# Autodesk Inventor assembly: Assembly v2
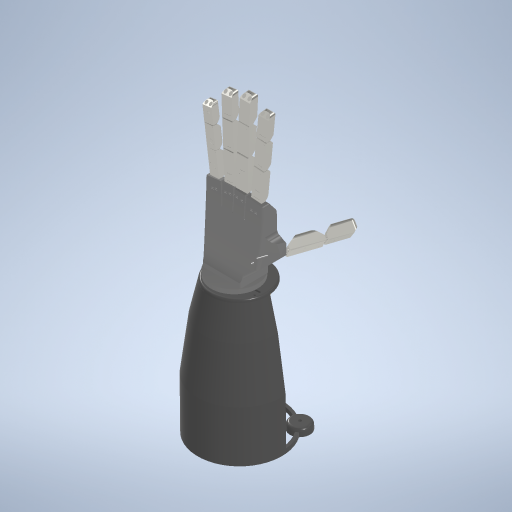
[picture p0: Inventor's stored thumbnail of the model, 512x512]
Saved by Autodesk Inventor 2024 (Build 280153000, 153)
## iProperties
Created: 2025-07-03
Part Number: Assembly v2
Document SubType Name: Assembly
Designer: Mehdi Charfeddine
Author: Mehdi Charfeddine
## Documents named in this file (15)
- C:\Users\Mehdi Charfeddine\OneDrive\Bureau\original 3d\Assembly v2.iam
- C:\Users\Mehdi Charfeddine\OneDrive\Bureau\original 3d\hand update v2.ipt
- C:\Users\Mehdi Charfeddine\OneDrive\Bureau\original 3d\update arm.ipt
- C:\Users\Mehdi Charfeddine\OneDrive\Bureau\original 3d\plaque motor.ipt
- C:\Users\Mehdi Charfeddine\OneDrive\Bureau\original 3d\finger\Daumen lower.ipt
- C:\Users\Mehdi Charfeddine\OneDrive\Bureau\original 3d\finger\Mittelfinger lower.ipt
- C:\Users\Mehdi Charfeddine\OneDrive\Bureau\original 3d\finger\Mittelfinger middle.ipt
- C:\Users\Mehdi Charfeddine\OneDrive\Bureau\original 3d\finger\Daumen upper.ipt
- C:\Users\Mehdi Charfeddine\OneDrive\Bureau\original 3d\finger\Mittelfinger upper.ipt
- C:\Users\Mehdi Charfeddine\OneDrive\Bureau\original 3d\finger\Ringfinger lower.ipt
- C:\Users\Mehdi Charfeddine\OneDrive\Bureau\original 3d\finger\Ringfinger middle.ipt
- C:\Users\Mehdi Charfeddine\OneDrive\Bureau\original 3d\finger\Ringfinger upper.ipt
- C:\Users\Mehdi Charfeddine\OneDrive\Bureau\original 3d\finger\Kleiner Finger lower.ipt
- C:\Users\Mehdi Charfeddine\OneDrive\Bureau\original 3d\finger\Kleiner Finger middle.ipt
- C:\Users\Mehdi Charfeddine\OneDrive\Bureau\original 3d\finger\Kleiner Finger upper.ipt
## Components (17 placed, 14 different names)
1. hand update v2:1 — Mate:1, Mate:3, Mate:4, Mate:8, Mate:10, Mate:14
2. update arm:1 — Mate:1, Mate:2
3. plaque motor:1 — Mate:2
4. Daumen lower:1 — Mate:3, Mate:5
5. Mittelfinger lower:1 — Mate:4, Mate:6
6. Mittelfinger middle:1 — Mate:6, Mate:7
7. Daumen upper:1 — Mate:5
8. Mittelfinger upper:1 — Mate:7
9. Ringfinger lower:1 — Mate:10, Mate:11
10. Ringfinger lower:2 — Mate:8, Mate:9
11. Ringfinger middle:1 — Mate:11, Mate:13
12. Ringfinger middle:2 — Mate:9, Mate:12
13. Ringfinger upper:1 — Mate:12
14. Ringfinger upper:2 — Mate:13
15. Kleiner Finger lower:1 — Mate:14, Mate:15
16. Kleiner Finger middle:1 — Mate:15, Mate:16
17. Kleiner Finger upper:1 — Mate:16
## Relationships (16: Mate 16)
- Mate:1: hand update v2:1 ↔ update arm:1
- Mate:2: update arm:1 ↔ plaque motor:1
- Mate:3: hand update v2:1 ↔ Daumen lower:1
- Mate:4: hand update v2:1 ↔ Mittelfinger lower:1
- Mate:5: Daumen lower:1 ↔ Daumen upper:1
- Mate:6: Mittelfinger lower:1 ↔ Mittelfinger middle:1
- Mate:7: Mittelfinger middle:1 ↔ Mittelfinger upper:1
- Mate:8: hand update v2:1 ↔ Ringfinger lower:2
- Mate:9: Ringfinger lower:2 ↔ Ringfinger middle:2
- Mate:10: hand update v2:1 ↔ Ringfinger lower:1
- Mate:11: Ringfinger lower:1 ↔ Ringfinger middle:1
- Mate:12: Ringfinger middle:2 ↔ Ringfinger upper:1
- Mate:13: Ringfinger middle:1 ↔ Ringfinger upper:2
- Mate:14: hand update v2:1 ↔ Kleiner Finger lower:1
- Mate:15: Kleiner Finger lower:1 ↔ Kleiner Finger middle:1
- Mate:16: Kleiner Finger middle:1 ↔ Kleiner Finger upper:1
